# Autodesk Inventor assembly: Assembly1
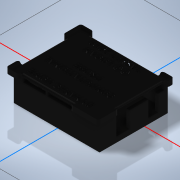
[picture p0: Inventor's stored thumbnail of the model, 180x180]
Saved by Autodesk Inventor 2020.1 (Build 241239000, 239)
## iProperties
Created: 2019-09-15
Part Number: Assembly1
Document SubType Name: Assembly
Designer: Logan
Author: Logan
## Documents named in this file (3)
- C:\Users\Logan\Desktop\Assembly1.iam
- C:\Users\Logan\Desktop\UNO Case.ipt
- C:\Users\Logan\Desktop\UNO Cover.ipt
## Components (2 placed, 2 different names)
1. UNO Case:1 — Mate:1
2. UNO Cover:1 — Mate:1
## Relationships (1: Mate 1)
- Mate:1: UNO Case:1 ↔ UNO Cover:1
